# Autodesk Inventor assembly: scara2
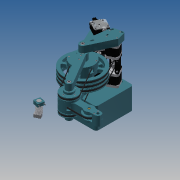
[picture p0: Inventor's stored thumbnail of the model, 180x180]
Saved by Autodesk Inventor 2013 (Build 170138000, 138)
## iProperties
Created: 2017-03-31
Part Number: scara2
Document SubType Name: Assembly
Designer: employee
Author: employee
## Documents named in this file (44)
- C:\Users\employee\Desktop\SCARA\scara2.iam
- C:\Users\employee\Desktop\SCARA\top plate.ipt
- C:\Users\employee\Desktop\SCARA\stepper.ipt
- C:\Users\employee\Desktop\SCARA\dual stepper mount.ipt
- C:\Users\employee\Desktop\SCARA\washer.ipt
- C:\Users\employee\Desktop\SCARA\drive pulley.ipt
- C:\Users\employee\Desktop\SCARA\driven arm.ipt
- C:\Users\employee\Desktop\SCARA\608 bearing.ipt
- C:\Users\employee\Desktop\SCARA\offset shield.ipt
- C:\Users\employee\Desktop\SCARA\M3x30.ipt
- C:\Users\employee\Desktop\SCARA\235 drive pulley.ipt
- C:\Users\employee\Desktop\SCARA\M3x60.ipt
- C:\Users\employee\Desktop\SCARA\M3x35.ipt
- C:\Users\employee\Desktop\SCARA\M3x8.ipt
- C:\Users\employee\Desktop\SCARA\bottom plate.ipt
- C:\Users\employee\Desktop\SCARA\distal idler pulley.ipt
- C:\Users\employee\Desktop\SCARA\z idler pulley.ipt
- C:\Users\employee\Desktop\SCARA\proximal thin arm.ipt
- C:\Users\employee\Desktop\SCARA\central pivot spacer.ipt
- C:\Users\employee\Desktop\SCARA\distal drive pulley.ipt
- C:\Users\employee\Desktop\SCARA\heat block.ipt
- C:\Users\employee\Desktop\SCARA\heat sink.ipt
- C:\Users\employee\Desktop\SCARA\nozzle.ipt
- C:\Users\employee\Desktop\SCARA\e3d mount.ipt
- C:\Users\employee\Desktop\SCARA\M3x45.ipt
- C:\Users\employee\Desktop\SCARA\M3x65.ipt
- C:\Users\employee\Desktop\SCARA\Imported Components\175_filament_feed\175_filament_feed.ipt
- C:\Users\employee\Desktop\SCARA\Imported Components\big_gear\big_gear.ipt
- C:\Users\employee\Desktop\SCARA\Imported Components\cilindar_fitting\cilindar_fitting.ipt
- C:\Users\employee\Desktop\SCARA\Imported Components\e3d extruder\e3d extruder.ipt
- C:\Users\employee\Desktop\SCARA\Imported Components\gornji dio e3d extruder\gornji dio e3d extruder.ipt
- C:\Users\employee\Desktop\SCARA\Imported Components\polugica\polugica.ipt
- C:\Users\employee\Desktop\SCARA\Imported Components\small gear\small gear.ipt
- C:\Users\employee\Desktop\SCARA\M3x25.ipt
- C:\Users\employee\Desktop\SCARA\first belt.ipt
- C:\Users\employee\Desktop\SCARA\middle belt.ipt
- C:\Users\employee\Desktop\SCARA\end belt.ipt
- C:\Users\employee\Desktop\SCARA\M8x120.ipt
- C:\Users\employee\Desktop\SCARA\M8x200.ipt
- C:\Users\employee\Desktop\SCARA\SCREW BOTTOM ARM.ipt
- C:\Users\employee\Desktop\SCARA\SCREW TOP ARM.ipt
- C:\Users\employee\Desktop\SCARA\SCREW Z IDLER.ipt
- C:\Users\employee\Desktop\SCARA\Z belt.ipt
- C:\Users\employee\Desktop\SCARA\screw nut.iam
## Components (105 placed, 43 different names)
1. top plate:1 — Insert:1, Insert:2, Insert:3, Insert:4, Insert:9, Insert:97, Insert:98, Insert:99, Insert:100, Insert:101, Insert:129
2. stepper:1 — Insert:2, Insert:3, Insert:7, Insert:8, Angle:2, Mate:14
3. stepper:2 — Insert:1, Insert:4, Insert:5, Insert:6, Insert:15
4. dual stepper mount:1 — Insert:5, Insert:6, Insert:12, Insert:13, Flush:1, Insert:28, Insert:29, Insert:30, Insert:34, Insert:35, Insert:36
5. dual stepper mount:2 — Insert:7, Insert:8, Insert:10, Insert:11, Insert:31, Insert:32, Insert:33, Insert:37, Insert:38, Insert:39
6. washer:1 — Insert:9, Insert:17
7. stepper:3 — Insert:10, Insert:11, Mate:1, Insert:41, Mate:17
8. stepper:4 — Insert:12, Insert:13, Insert:14, Insert:40
9. drive pulley:1 — Flush:1, Mate:1
10. drive pulley:2 — Insert:15, Mate:19
11. drive pulley:3 — Insert:14, Mate:18
12. driven arm:1 — Insert:16, Insert:19, Insert:22, Insert:24, Mate:3, Insert:59, Insert:130
13. 608 bearing:2 — Insert:16, Insert:17
14. offset shield:1 — Insert:19, Insert:20, Insert:25, Insert:26, Insert:27, Insert:46, Insert:47
15. 608 bearing:3 — Insert:20, Insert:21
16. washer:2 — Insert:21, Insert:44
17. M3x30:1 — Insert:22
18. 235 drive pulley:1 — Insert:46, Insert:47, Insert:111
19. M3x60:1 — Insert:24
20. M3x35:1 — Insert:25
21. M3x35:2 — Insert:26
22. M3x35:3 — Insert:27
23. M3x8:1 — Insert:33
24. M3x8:2 — Insert:28
25. M3x8:3 — Insert:29
26. M3x8:4 — Insert:31
27. M3x8:5 — Insert:32
28. M3x8:6 — Insert:30
29. M3x8:7 — Insert:36
30. M3x8:8 — Insert:35
31. M3x8:9 — Insert:34
32. M3x8:10 — Insert:37
33. M3x8:11 — Insert:38
34. M3x8:12 — Insert:39
35. bottom plate:1 — Insert:40, Insert:41, Insert:89, Insert:90, Insert:91, Insert:92, Insert:93, Insert:94, Insert:95, Insert:96, z, y, x
36. distal idler pulley:1 — Insert:42, Insert:43, Insert:112, Insert:115
37. 608 bearing:4 — Insert:42, Insert:44
38. 608 bearing:5 — Insert:43, Insert:45
39. washer:3 — Insert:45, Insert:50
40. z idler pulley:2 — Insert:48, Insert:49, Insert:113, Insert:114
41. 608 bearing:6 — Insert:48, Insert:51
42. 608 bearing:7 — Insert:49, Insert:50
43. washer:4 — Insert:51, Insert:54
44. proximal thin arm:1 — Insert:52, Insert:53, Mate:3, Insert:60, Mate:20
45. 608 bearing:8 — Insert:53, Insert:54
46. 608 bearing:9 — Insert:52, Insert:55
47. washer:5 — Insert:55, Insert:88
48. central pivot spacer:1 — Insert:88
49. washer:6 — Insert:59, Insert:62
50. washer:7 — Insert:60
51. distal drive pulley:1 — Insert:61, Insert:66, Insert:67, Insert:68, Insert:69, Mate:21, Insert:131
52. 608 bearing:10 — Insert:61, Insert:62
53. M3x30:2 — Insert:66
54. M3x30:3 — Insert:67, Mate:24
55. M3x30:4 — Insert:68
56. M3x30:5 — Insert:69
57. heat block:1 — Insert:84
58. heat sink:1 — Insert:84, Insert:85, Mate:8, Mate:9, Mate:12
59. nozzle:1 — Insert:85, z, y, x
60. e3d mount:1 — Mate:8, Mate:10
61. e3d mount:2 — Mate:9, Mate:10, Mate:12, Insert:86, Insert:87
62. M3x30:6 — Insert:86
63. M3x30:7 — Insert:87
64. M3x45:1 — Insert:96
65. M3x45:2 — Insert:95
66. M3x45:3 — Insert:93
67. M3x45:4 — Insert:91
68. M3x45:5 — Insert:90
69. M3x45:6 — Insert:89
70. M3x45:7 — Insert:92
71. M3x45:8 — Insert:94
72. M3x65:1 — Insert:97
73. M3x65:2 — Insert:99
74. M3x65:3 — Insert:100
75. M3x65:4 — Insert:98
76. 175_filament_feed:1 — Insert:102, Angle:3
77. big_gear:1 — Insert:105
78. cilindar_fitting:1 — Insert:103
79. e3d extruder:1 — Insert:101, Angle:2, Insert:102, Angle:3, Mate:15, Angle:4, Insert:103, Insert:105, Insert:106, Angle:5
80. gornji dio e3d extruder:1 — Insert:106, Angle:5, Insert:107, Insert:108, Insert:109, Insert:110
81. polugica:1 — Mate:14, Mate:16, Insert:104
82. small gear:1 — Insert:104
83. M3x35:4 — Insert:107
84. M3x35:5 — Insert:108
85. M3x35:6 — Insert:109
86. M3x25:1 — Insert:110
87. first belt:1 — Insert:111, Mate:19
88. first belt:2 — Insert:112, Mate:17
89. first belt:3 — Insert:113, Mate:18
90. middle belt:1 — Insert:114, Mate:20
91. middle belt:2 — Insert:115, Mate:21
92. end belt:1
93. M8x120:1 — Insert:130
94. M8x200:1 — Insert:129
95. SCREW BOTTOM ARM:1 — Insert:134, Insert:135
96. SCREW TOP ARM:1 — Insert:131, Mate:24, Insert:132, Insert:134, Insert:135, Mate:25, Insert:140, Insert:141, Insert:142
97. 608 bearing:11 — Insert:132, Insert:133
98. washer:8 — Insert:133, Insert:138
99. SCREW Z IDLER:1 — Insert:136, Insert:137, Insert:139
100. 608 bearing:12 — Insert:136, Insert:138
101. 608 bearing:13 — Insert:137
102. Z belt:1 — Insert:139, Mate:25
103. screw nut:1 [sub-assembly] — Insert:140
104. M3x35:7 — Insert:142
105. M3x35:8 — Insert:141
## Relationships (131: Insert 107, Mate 18, Angle 4, Flush 2)
- Insert:1: top plate:1 ↔ stepper:2
- Insert:2: top plate:1 ↔ stepper:1
- Insert:3: top plate:1 ↔ stepper:1
- Insert:4: top plate:1 ↔ stepper:2
- Insert:5: stepper:2 ↔ dual stepper mount:1
- Insert:6: stepper:2 ↔ dual stepper mount:1
- Insert:7: stepper:1 ↔ dual stepper mount:2
- Insert:8: stepper:1 ↔ dual stepper mount:2
- Insert:9: top plate:1 ↔ washer:1
- Insert:10: dual stepper mount:2 ↔ stepper:3
- Insert:11: dual stepper mount:2 ↔ stepper:3
- Insert:12: dual stepper mount:1 ↔ stepper:4
- Insert:13: dual stepper mount:1 ↔ stepper:4
- Insert:14 (3.75 mm): stepper:4 ↔ drive pulley:3
- Insert:15 (3.5 mm): stepper:2 ↔ drive pulley:2
- Flush:1: dual stepper mount:1 ↔ drive pulley:1
- Mate:1: stepper:3 ↔ drive pulley:1
- Insert:16: driven arm:1 ↔ 608 bearing:2
- Insert:17: washer:1 ↔ 608 bearing:2
- Insert:19: driven arm:1 ↔ offset shield:1
- Insert:20: offset shield:1 ↔ 608 bearing:3
- Insert:21: 608 bearing:3 ↔ washer:2
- Insert:22: driven arm:1 ↔ M3x30:1
- Insert:24: driven arm:1 ↔ M3x60:1
- Insert:25: offset shield:1 ↔ M3x35:1
- Insert:26: offset shield:1 ↔ M3x35:2
- Insert:27: offset shield:1 ↔ M3x35:3
- Insert:28: dual stepper mount:1 ↔ M3x8:2
- Insert:29: dual stepper mount:1 ↔ M3x8:3
- Insert:30: dual stepper mount:1 ↔ M3x8:6
- Insert:31: dual stepper mount:2 ↔ M3x8:4
- Insert:32: dual stepper mount:2 ↔ M3x8:5
- Insert:33: dual stepper mount:2 ↔ M3x8:1
- Insert:34: dual stepper mount:1 ↔ M3x8:9
- Insert:35: dual stepper mount:1 ↔ M3x8:8
- Insert:36: dual stepper mount:1 ↔ M3x8:7
- Insert:37: dual stepper mount:2 ↔ M3x8:10
- Insert:38: dual stepper mount:2 ↔ M3x8:11
- Insert:39: dual stepper mount:2 ↔ M3x8:12
- Insert:40: stepper:4 ↔ bottom plate:1
- Insert:41: stepper:3 ↔ bottom plate:1
- Insert:42: distal idler pulley:1 ↔ 608 bearing:4
- Insert:43: distal idler pulley:1 ↔ 608 bearing:5
- Insert:44: washer:2 ↔ 608 bearing:4
- Insert:45: 608 bearing:5 ↔ washer:3
- Insert:46: offset shield:1 ↔ 235 drive pulley:1
- Insert:47: offset shield:1 ↔ 235 drive pulley:1
- Insert:48: z idler pulley:2 ↔ 608 bearing:6
- Insert:49: z idler pulley:2 ↔ 608 bearing:7
- Insert:50: washer:3 ↔ 608 bearing:7
- Insert:51: 608 bearing:6 ↔ washer:4
- Insert:52: proximal thin arm:1 ↔ 608 bearing:9
- Insert:53: proximal thin arm:1 ↔ 608 bearing:8
- Insert:54: washer:4 ↔ 608 bearing:8
- Insert:55: 608 bearing:9 ↔ washer:5
- Mate:3: driven arm:1 ↔ proximal thin arm:1
- Insert:59: driven arm:1 ↔ washer:6
- Insert:60: proximal thin arm:1 ↔ washer:7
- Insert:61: distal drive pulley:1 ↔ 608 bearing:10
- Insert:62: washer:6 ↔ 608 bearing:10
- Insert:66: distal drive pulley:1 ↔ M3x30:2
- Insert:67: distal drive pulley:1 ↔ M3x30:3
- Insert:68: distal drive pulley:1 ↔ M3x30:4
- Insert:69: distal drive pulley:1 ↔ M3x30:5
- Insert:84: heat block:1 ↔ heat sink:1
- Insert:85: heat sink:1 ↔ nozzle:1
- Mate:8: heat sink:1 ↔ e3d mount:1
- Mate:9: heat sink:1 ↔ e3d mount:2
- Mate:10: e3d mount:1 ↔ e3d mount:2
- Mate:12: heat sink:1 ↔ e3d mount:2
- Insert:86: e3d mount:2 ↔ M3x30:6
- Insert:87: e3d mount:2 ↔ M3x30:7
- Insert:88: washer:5 ↔ central pivot spacer:1
- Insert:89: bottom plate:1 ↔ M3x45:6
- Insert:90: bottom plate:1 ↔ M3x45:5
- Insert:91: bottom plate:1 ↔ M3x45:4
- Insert:92: bottom plate:1 ↔ M3x45:7
- Insert:93: bottom plate:1 ↔ M3x45:3
- Insert:94: bottom plate:1 ↔ M3x45:8
- Insert:95: bottom plate:1 ↔ M3x45:2
- Insert:96: bottom plate:1 ↔ M3x45:1
- Insert:97: top plate:1 ↔ M3x65:1
- Insert:98: top plate:1 ↔ M3x65:4
- Insert:99: top plate:1 ↔ M3x65:2
- Insert:100: top plate:1 ↔ M3x65:3
- Insert:101: top plate:1 ↔ e3d extruder:1
- Angle:2 (0 deg): stepper:1 ↔ e3d extruder:1
- Insert:102: 175_filament_feed:1 ↔ e3d extruder:1
- Angle:3 (0 deg): 175_filament_feed:1 ↔ e3d extruder:1
- Mate:14: stepper:1 ↔ polugica:1
- Mate:15: e3d extruder:1
- Angle:4 (0 deg): e3d extruder:1
- Mate:16: polugica:1
- Insert:103: cilindar_fitting:1 ↔ e3d extruder:1
- Insert:104: polugica:1 ↔ small gear:1
- Insert:105: big_gear:1 ↔ e3d extruder:1
- Insert:106: e3d extruder:1 ↔ gornji dio e3d extruder:1
- Angle:5 (0 deg): e3d extruder:1 ↔ gornji dio e3d extruder:1
- Insert:107: gornji dio e3d extruder:1 ↔ M3x35:4
- Insert:108: gornji dio e3d extruder:1 ↔ M3x35:5
- Insert:109: gornji dio e3d extruder:1 ↔ M3x35:6
- Insert:110: gornji dio e3d extruder:1 ↔ M3x25:1
- Insert:111 (1 mm): 235 drive pulley:1 ↔ first belt:1
- Insert:112 (1 mm): distal idler pulley:1 ↔ first belt:2
- Insert:113 (1 mm): z idler pulley:2 ↔ first belt:3
- Mate:17: stepper:3 ↔ first belt:2
- Mate:18: drive pulley:3 ↔ first belt:3
- Mate:19: drive pulley:2 ↔ first belt:1
- Insert:114 (1 mm): z idler pulley:2 ↔ middle belt:1
- Insert:115 (1 mm): distal idler pulley:1 ↔ middle belt:2
- Mate:20: proximal thin arm:1 ↔ middle belt:1
- Mate:21: distal drive pulley:1 ↔ middle belt:2
- z [Flush] (-10 mm): bottom plate:1 ↔ nozzle:1
- y [Mate] (79 mm): bottom plate:1 ↔ nozzle:1
- x [Mate]: bottom plate:1 ↔ nozzle:1
- Insert:129: top plate:1 ↔ M8x200:1
- Insert:130: driven arm:1 ↔ M8x120:1
- Insert:131: distal drive pulley:1 ↔ SCREW TOP ARM:1
- Mate:24: M3x30:3 ↔ SCREW TOP ARM:1
- Insert:132: SCREW TOP ARM:1 ↔ 608 bearing:11
- Insert:133: 608 bearing:11 ↔ washer:8
- Insert:134: SCREW BOTTOM ARM:1 ↔ SCREW TOP ARM:1
- Insert:135: SCREW BOTTOM ARM:1 ↔ SCREW TOP ARM:1
- Insert:136: SCREW Z IDLER:1 ↔ 608 bearing:12
- Insert:137: SCREW Z IDLER:1 ↔ 608 bearing:13
- Insert:138: washer:8 ↔ 608 bearing:12
- Insert:139 (1 mm): SCREW Z IDLER:1 ↔ Z belt:1
- Mate:25: SCREW TOP ARM:1 ↔ Z belt:1
- Insert:140: SCREW TOP ARM:1 ↔ screw nut:1
- Insert:141: SCREW TOP ARM:1 ↔ M3x35:8
- Insert:142: SCREW TOP ARM:1 ↔ M3x35:7
## Named parameters: z = 10 mm, x = 75 mm, y = 100 mm
